# Autodesk Inventor assembly: Ajedrez2
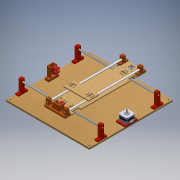
[picture p0: Inventor's stored thumbnail of the model, 180x180]
Saved by Autodesk Inventor 2019 (Build 230136000, 136)
## iProperties
Created: 2019-08-18
Part Number: Ajedrez2
Document SubType Name: Assembly
Designer: Bruno
Author: Bruno
## Documents named in this file (9)
- C:\Users\Bruno\Stuff\TPINFO\tp-info\Ajedrez2.iam
- C:\Users\Bruno\Stuff\TPINFO\tp-info\Floor.ipt
- C:\Users\Bruno\Stuff\TPINFO\tp-info\XRodClamp.ipt
- C:\Users\Bruno\Stuff\TPINFO\tp-info\XRod.ipt
- C:\Users\Bruno\Stuff\TPINFO\tp-info\XMotor.iam
- C:\Users\Bruno\Stuff\TPINFO\tp-info\XPulleySupport.iam
- C:\Users\Bruno\Stuff\TPINFO\tp-info\XCart.iam
- C:\Users\Bruno\Stuff\TPINFO\tp-info\YCart.iam
- C:\Users\Bruno\Stuff\TPINFO\tp-info\Lid.iam
## Components (12 placed, 8 different names)
1. Floor:1 — Rigid:1, Rigid:2, Rigid:3, Rigid:4, Rigid:7, Rigid:8, Flush:1, Flush:2
2. XRodClamp:1 — Rigid:1, Rigid:5
3. XRodClamp:2 — Rigid:2
4. XRodClamp:3 — Rigid:3, Rigid:6
5. XRodClamp:4 — Rigid:4
6. XRod:1 — Rigid:5, Cylindrical:2
7. XRod:2 — Rigid:6, Cylindrical:1
8. XMotor:1 [sub-assembly] — Rigid:7
9. XPulleySupport:1 [sub-assembly] — Rigid:8
10. XCart:1 [sub-assembly] — Cylindrical:1, Cylindrical:2, Cylindrical:3
11. YCart:1 [sub-assembly] — Cylindrical:3
12. Lid:1 [sub-assembly] — Flush:1, Flush:2
## Relationships (13: WeldJoint 8, CylindricalJoint 3, Flush 2)
- Rigid:1 [WeldJoint]: Floor:1 ↔ XRodClamp:1
- Rigid:2 [WeldJoint]: Floor:1 ↔ XRodClamp:2
- Rigid:3 [WeldJoint]: Floor:1 ↔ XRodClamp:3
- Rigid:4 [WeldJoint]: Floor:1 ↔ XRodClamp:4
- Rigid:5 [WeldJoint]: XRodClamp:1 ↔ XRod:1
- Rigid:6 [WeldJoint]: XRodClamp:3 ↔ XRod:2
- Rigid:7 [WeldJoint]: Floor:1 ↔ XMotor:1
- Rigid:8 [WeldJoint]: Floor:1 ↔ XPulleySupport:1
- Cylindrical:1: XRod:2 ↔ XCart:1
- Cylindrical:2: XRod:1 ↔ XCart:1
- Cylindrical:3: XCart:1 ↔ YCart:1
- Flush:1: Floor:1 ↔ Lid:1
- Flush:2: Floor:1 ↔ Lid:1
